# Autodesk Inventor assembly: Assembly1
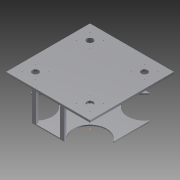
[picture p0: Inventor's stored thumbnail of the model, 180x180]
Saved by Autodesk Inventor 2011 (Build 150239000, 239)
## iProperties
Created: 2011-08-21
Part Number: Assembly1
Document SubType Name: Assembly
Designer: Matthew
Author: Matthew
## Documents named in this file (4)
- C:\Users\Matthew\Documents\matthew_autocad\prlite\base\BASE.iam
- C:\Users\Matthew\Documents\matthew_autocad\prlite\base\base top.ipt
- C:\Users\Matthew\Documents\matthew_autocad\prlite\base\base bottom.ipt
- C:\Users\Matthew\Documents\matthew_autocad\prlite\base\top-bot connector lame.ipt
## Components (10 placed, 3 different names)
1. base top:1 — Flush:14, Mate:2, Mate:6, Flush:19, Mate:7, Mate:8, Mate:10, Flush:22, Mate:11, Flush:24, Flush:25, Flush:26, Mate:12, Flush:29, Flush:30, Flush:31, Mate:13, Flush:34
2. base bottom:1 — Flush:17, Flush:20, Mate:9, Flush:21, Flush:23, Flush:27, Flush:28, Flush:32, Flush:33
3. top-bot connector lame:2 — Flush:14, Mate:2, Flush:17, Mate:7
4. top-bot connector lame:3 — Mate:6, Flush:19, Mate:8, Flush:20, Mate:9
5. top-bot connector lame:4 — Flush:33, Mate:13, Flush:34
6. top-bot connector lame:5 — Flush:30, Flush:31, Flush:32
7. top-bot connector lame:6 — Mate:12, Flush:28, Flush:29
8. top-bot connector lame:7 — Flush:25, Flush:26, Flush:27
9. top-bot connector lame:8 — Mate:10, Flush:21, Flush:22
10. top-bot connector lame:9 — Flush:23, Mate:11, Flush:24
## Relationships (27: Flush 18, Mate 9)
- Flush:14: base top:1 ↔ top-bot connector lame:2
- Mate:2: base top:1 ↔ top-bot connector lame:2
- Flush:17: base bottom:1 ↔ top-bot connector lame:2
- Mate:6: base top:1 ↔ top-bot connector lame:3
- Flush:19: base top:1 ↔ top-bot connector lame:3
- Mate:7: base top:1 ↔ top-bot connector lame:2
- Mate:8: base top:1 ↔ top-bot connector lame:3
- Flush:20: base bottom:1 ↔ top-bot connector lame:3
- Mate:9: base bottom:1 ↔ top-bot connector lame:3
- Mate:10: base top:1 ↔ top-bot connector lame:8
- Flush:21: base bottom:1 ↔ top-bot connector lame:8
- Flush:22: base top:1 ↔ top-bot connector lame:8
- Flush:23: base bottom:1 ↔ top-bot connector lame:9
- Mate:11: base top:1 ↔ top-bot connector lame:9
- Flush:24: base top:1 ↔ top-bot connector lame:9
- Flush:25: base top:1 ↔ top-bot connector lame:7
- Flush:26: base top:1 ↔ top-bot connector lame:7
- Flush:27: base bottom:1 ↔ top-bot connector lame:7
- Mate:12: base top:1 ↔ top-bot connector lame:6
- Flush:28: base bottom:1 ↔ top-bot connector lame:6
- Flush:29: base top:1 ↔ top-bot connector lame:6
- Flush:30: base top:1 ↔ top-bot connector lame:5
- Flush:31: base top:1 ↔ top-bot connector lame:5
- Flush:32: base bottom:1 ↔ top-bot connector lame:5
- Flush:33: base bottom:1 ↔ top-bot connector lame:4
- Mate:13: base top:1 ↔ top-bot connector lame:4
- Flush:34: base top:1 ↔ top-bot connector lame:4
